# Autodesk Inventor assembly: full door assembly
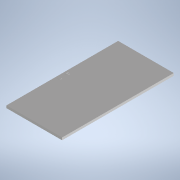
[picture p0: Inventor's stored thumbnail of the model, 180x180]
Saved by Autodesk Inventor 2022 (Build 260153000, 153)
## iProperties
Created: 2022-06-16
Part Number: full door assembly
Document SubType Name: Assembly
Designer: alecw
Author: alecw
## Documents named in this file (3)
- C:\aw_gd\Coding and Projects\smart home\smart-deadbolt\3D Modelling\full door assembly.iam
- C:\aw_gd\Coding and Projects\smart home\smart-deadbolt\3D Modelling\door.ipt
- C:\aw_gd\Coding and Projects\smart home\smart-deadbolt\3D Modelling\deadbolt arm.ipt
## Components (2 placed, 2 different names)
1. door:1 — Cylindrical:1, Mate:1, Mate:2
2. deadbolt arm:1 — Cylindrical:1, Mate:1
## Relationships (3: Mate 2, CylindricalJoint 1)
- Cylindrical:1: door:1 ↔ deadbolt arm:1
- Mate:1: door:1 ↔ deadbolt arm:1
- Mate:2: door:1
